# Autodesk Inventor assembly: Assy_cover_right
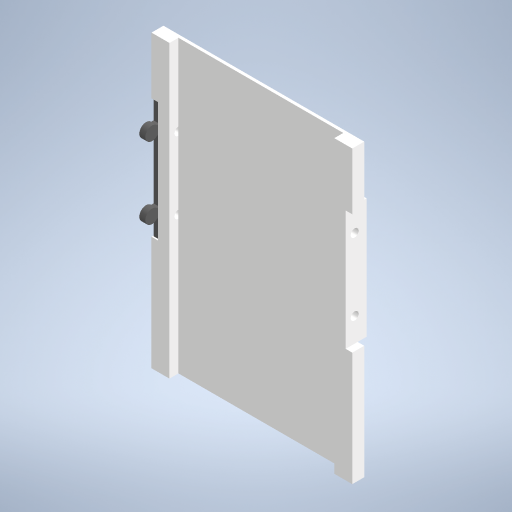
[picture p0: Inventor's stored thumbnail of the model, 512x512]
Saved by Autodesk Inventor 2024.1 (Build 281209000, 209)
## iProperties
Created: 2025-03-07
Part Number: Assy_cover_right
Document SubType Name: Assembly
Designer: hibik
Author: hibik
## Documents named in this file (3)
- C:\Users\hibik\Documents\Robomech\RESCUE\ORCA\hard\cover\Assy_cover_right.iam
- C:\Users\hibik\Documents\Robomech\RESCUE\ORCA\hard\cover\cover_right.ipt
- C:\Users\hibik\Documents\Robomech\RESCUE\ORCA\hard\cover\cover_setter.ipt
## Components (2 placed, 2 different names)
1. cover_right:1 — 挿入:1, 挿入:2
2. cover_setter:2 — 挿入:1, 挿入:2
## Relationships (2: Insert 2)
- 挿入:1 [Insert]: cover_right:1 ↔ cover_setter:2
- 挿入:2 [Insert]: cover_right:1 ↔ cover_setter:2
